# Autodesk Inventor assembly: Fully_made_PCB
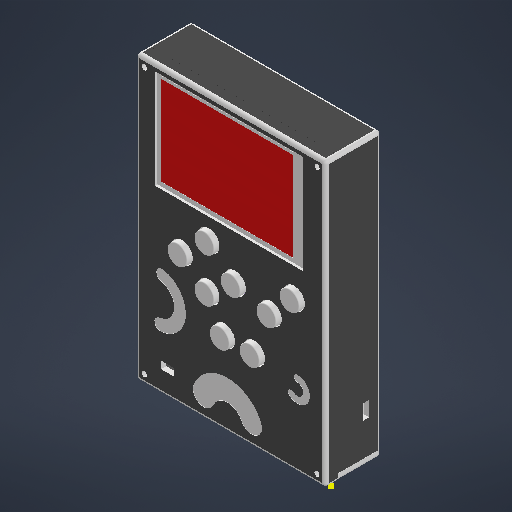
[picture p0: Inventor's stored thumbnail of the model, 512x512]
Saved by Autodesk Inventor 2026 (Build 300175050, 175E)
## iProperties
Created: 2025-07-08
Part Number: Fully_made_PCB
Document SubType Name: Assembly
Designer: SaiAn
Author: SaiAn
## Documents named in this file (10)
- C:\Retro Game Console\Fully_made_PCB.iam
- C:\Retro Game Console\raspberry-pi-zero-heatsink-1.snapshot.3\waveshare_PiZero_heatsink\waveshare_PiZero_heatsink\waveshare_PiZero_heatsink.ipt
- C:\Retro Game Console\waveshare-3-5-60fps-raspberry-pi-resistive-hdmi-lcd-display-480x320-ws12824-1.snapshot.3\Waveshare_HDMI_3,5_Zoll_Display\Waveshare_HDMI_3,5_Zoll_Display\Waveshare_HDMI_3,5_Zoll_Display.ipt
- C:\Retro Game Console\COC.ipt
- C:\Retro Game Console\RetroGameConsole\RetroGameConsole\RetroGameConsole\RetroGameConsole.ipt
- C:\Retro Game Console\RetroGameConsole\RetroGameConsole\Push_Button_6.2x6.2_2pins v1.ipt
- C:\Retro Game Console\raspberry-pi-zero-2-w-with-40-pin-male-connector-1.snapshot.2\Raspberry Pi Zero 2 W with 40 pin male connector v4\Raspberry Pi Zero 2 W with 40 pin male connector v4\Raspberry Pi Zero 2 W .ipt
- C:\Retro Game Console\adafruit-powerboost-1000-1.snapshot.4\powerboost 1000c.f3d v3\powerboost 1000c.f3d v3\powerboost 1000c.f3d v3.ipt
- C:\Retro Game Console\POC.ipt
- C:\Retro Game Console\THEREALBUTTON.ipt
## Components (23 placed, 9 different names)
1. RetroGameConsole:1 — Mate:1, Mate:2, Mate:3, Mate:4, Mate:5, Mate:6, Mate:7, Mate:8, Mate:9, Mate:10, Mate:11, Mate:12, Mate:13, Mate:14, Mate:15, Mate:16, Mate:17, Mate:18, Mate:19, Mate:20, Mate:21, Mate:22, Mate:23, Mate:24, Mate:25, Mate:26, Mate:27, Mate:28, Mate:29, Mate:33, Mate:34, Mate:35, Mate:36, Mate:37
2. Push_Button_6.2x6.2_2pins v1:1 — Mate:2, Mate:19, Mate:20, Mate:46, Mate:51
3. Push_Button_6.2x6.2_2pins v1:2 — Mate:5, Mate:11, Mate:12, Mate:49, Mate:56
4. Push_Button_6.2x6.2_2pins v1:3 — Mate:4, Mate:23, Mate:24, Mate:43, Mate:55
5. Push_Button_6.2x6.2_2pins v1:4 — Mate:6, Mate:17, Mate:18, Mate:45, Mate:58
6. Push_Button_6.2x6.2_2pins v1:5 — Mate:1, Mate:9, Mate:10, Mate:50, Mate:54
7. Push_Button_6.2x6.2_2pins v1:6 — Mate:3, Mate:21, Mate:22, Mate:44, Mate:57
8. Push_Button_6.2x6.2_2pins v1:7 — Mate:7, Mate:13, Mate:14, Mate:48, Mate:53
9. Push_Button_6.2x6.2_2pins v1:8 — Mate:8, Mate:15, Mate:16, Mate:47, Mate:52
10. Raspberry Pi Zero 2 W :1 — Mate:25, Mate:26, Mate:27, Mate:28, Mate:29, Mate:30, Mate:31, Mate:32, Mate:38, Flush:1, Flush:2
11. waveshare_PiZero_heatsink:1 — Mate:30, Mate:31, Mate:32
12. COC:1 — Mate:33, Mate:34, Mate:35, Mate:36, Mate:37, Mate:39, Mate:40, Mate:41, Mate:42, Flush:3, Flush:4
13. Waveshare_HDMI_3,5_Zoll_Display:1 — Mate:38, Flush:1, Flush:2
14. powerboost 1000c.f3d v3:2 — Mate:39, Mate:40
15. POC:1 — Mate:41, Mate:42, Flush:3, Flush:4
16. THEREALBUTTON:1 — Mate:43, Mate:55
17. THEREALBUTTON:2 — Mate:44, Mate:57
18. THEREALBUTTON:3 — Mate:46, Mate:51
19. THEREALBUTTON:4 — Mate:45, Mate:58
20. THEREALBUTTON:5 — Mate:50, Mate:54
21. THEREALBUTTON:6 — Mate:47, Mate:52
22. THEREALBUTTON:7 — Mate:48, Mate:53
23. THEREALBUTTON:8 — Mate:49, Mate:56
## Relationships (62: Mate 58, Flush 4)
- Mate:1: RetroGameConsole:1 ↔ Push_Button_6.2x6.2_2pins v1:5
- Mate:2: RetroGameConsole:1 ↔ Push_Button_6.2x6.2_2pins v1:1
- Mate:3: RetroGameConsole:1 ↔ Push_Button_6.2x6.2_2pins v1:6
- Mate:4: RetroGameConsole:1 ↔ Push_Button_6.2x6.2_2pins v1:3
- Mate:5: RetroGameConsole:1 ↔ Push_Button_6.2x6.2_2pins v1:2
- Mate:6: RetroGameConsole:1 ↔ Push_Button_6.2x6.2_2pins v1:4
- Mate:7: RetroGameConsole:1 ↔ Push_Button_6.2x6.2_2pins v1:7
- Mate:8: RetroGameConsole:1 ↔ Push_Button_6.2x6.2_2pins v1:8
- Mate:9: RetroGameConsole:1 ↔ Push_Button_6.2x6.2_2pins v1:5
- Mate:10: RetroGameConsole:1 ↔ Push_Button_6.2x6.2_2pins v1:5
- Mate:11: RetroGameConsole:1 ↔ Push_Button_6.2x6.2_2pins v1:2
- Mate:12: RetroGameConsole:1 ↔ Push_Button_6.2x6.2_2pins v1:2
- Mate:13: RetroGameConsole:1 ↔ Push_Button_6.2x6.2_2pins v1:7
- Mate:14: RetroGameConsole:1 ↔ Push_Button_6.2x6.2_2pins v1:7
- Mate:15: RetroGameConsole:1 ↔ Push_Button_6.2x6.2_2pins v1:8
- Mate:16: RetroGameConsole:1 ↔ Push_Button_6.2x6.2_2pins v1:8
- Mate:17: RetroGameConsole:1 ↔ Push_Button_6.2x6.2_2pins v1:4
- Mate:18: RetroGameConsole:1 ↔ Push_Button_6.2x6.2_2pins v1:4
- Mate:19: RetroGameConsole:1 ↔ Push_Button_6.2x6.2_2pins v1:1
- Mate:20: RetroGameConsole:1 ↔ Push_Button_6.2x6.2_2pins v1:1
- Mate:21: RetroGameConsole:1 ↔ Push_Button_6.2x6.2_2pins v1:6
- Mate:22: RetroGameConsole:1 ↔ Push_Button_6.2x6.2_2pins v1:6
- Mate:23: RetroGameConsole:1 ↔ Push_Button_6.2x6.2_2pins v1:3
- Mate:24: RetroGameConsole:1 ↔ Push_Button_6.2x6.2_2pins v1:3
- Mate:25: RetroGameConsole:1 ↔ Raspberry Pi Zero 2 W :1
- Mate:26: RetroGameConsole:1 ↔ Raspberry Pi Zero 2 W :1
- Mate:27: RetroGameConsole:1 ↔ Raspberry Pi Zero 2 W :1
- Mate:28: RetroGameConsole:1 ↔ Raspberry Pi Zero 2 W :1
- Mate:29: RetroGameConsole:1 ↔ Raspberry Pi Zero 2 W :1
- Mate:30: Raspberry Pi Zero 2 W :1 ↔ waveshare_PiZero_heatsink:1
- Mate:31: Raspberry Pi Zero 2 W :1 ↔ waveshare_PiZero_heatsink:1
- Mate:32: Raspberry Pi Zero 2 W :1 ↔ waveshare_PiZero_heatsink:1
- Mate:33: RetroGameConsole:1 ↔ COC:1
- Mate:34: RetroGameConsole:1 ↔ COC:1
- Mate:35: RetroGameConsole:1 ↔ COC:1
- Mate:36: RetroGameConsole:1 ↔ COC:1
- Mate:37: RetroGameConsole:1 ↔ COC:1
- Mate:38: Raspberry Pi Zero 2 W :1 ↔ Waveshare_HDMI_3,5_Zoll_Display:1
- Flush:1: Raspberry Pi Zero 2 W :1 ↔ Waveshare_HDMI_3,5_Zoll_Display:1
- Flush:2: Raspberry Pi Zero 2 W :1 ↔ Waveshare_HDMI_3,5_Zoll_Display:1
- Mate:39: COC:1 ↔ powerboost 1000c.f3d v3:2
- Mate:40: COC:1 ↔ powerboost 1000c.f3d v3:2
- Mate:41: COC:1 ↔ POC:1
- Mate:42: COC:1 ↔ POC:1
- Flush:3: COC:1 ↔ POC:1
- Flush:4: COC:1 ↔ POC:1
- Mate:43: Push_Button_6.2x6.2_2pins v1:3 ↔ THEREALBUTTON:1
- Mate:44: Push_Button_6.2x6.2_2pins v1:6 ↔ THEREALBUTTON:2
- Mate:45: Push_Button_6.2x6.2_2pins v1:4 ↔ THEREALBUTTON:4
- Mate:46: Push_Button_6.2x6.2_2pins v1:1 ↔ THEREALBUTTON:3
- Mate:47: Push_Button_6.2x6.2_2pins v1:8 ↔ THEREALBUTTON:6
- Mate:48: Push_Button_6.2x6.2_2pins v1:7 ↔ THEREALBUTTON:7
- Mate:49: Push_Button_6.2x6.2_2pins v1:2 ↔ THEREALBUTTON:8
- Mate:50: Push_Button_6.2x6.2_2pins v1:5 ↔ THEREALBUTTON:5
- Mate:51: Push_Button_6.2x6.2_2pins v1:1 ↔ THEREALBUTTON:3
- Mate:52: Push_Button_6.2x6.2_2pins v1:8 ↔ THEREALBUTTON:6
- Mate:53: Push_Button_6.2x6.2_2pins v1:7 ↔ THEREALBUTTON:7
- Mate:54: Push_Button_6.2x6.2_2pins v1:5 ↔ THEREALBUTTON:5
- Mate:55: Push_Button_6.2x6.2_2pins v1:3 ↔ THEREALBUTTON:1
- Mate:56: Push_Button_6.2x6.2_2pins v1:2 ↔ THEREALBUTTON:8
- Mate:57: Push_Button_6.2x6.2_2pins v1:6 ↔ THEREALBUTTON:2
- Mate:58: Push_Button_6.2x6.2_2pins v1:4 ↔ THEREALBUTTON:4
## Named parameters: Finish1_Area = 38.8096, Finish1_Thickness = 0.05 mm
note: some values were not read from the file. Shown as the stored number, unit unknown: "Finish1_Area".
